# Autodesk Inventor assembly: 000.002 - Крепеж мотора СБ
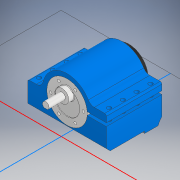
[picture p0: Inventor's stored thumbnail of the model, 180x180]
Saved by Autodesk Inventor 2022 (Build 260153000, 153)
## iProperties
Created: 2022-02-23
Part Number: 000.002 - Крепеж мотора СБ
Document SubType Name: Assembly
Designer: Petrov Ivan
Author: Petrov Ivan
## Documents named in this file (8)
- D:\IVAN\Ivan_desktop\Kvantorium\Projects\YouBotRobot\design\000.002 - Крепеж мотора СБ.iam
- D:\IVAN\Ivan_desktop\Kvantorium\Projects\YouBotRobot\design\000.002.001 - Крепеж мотора.ipt
- D:\IVAN\Ivan_desktop\Kvantorium\Projects\YouBotRobot\design\standart_components\dc_gear_motor_12V_500rpm.ipt
- D:\IVAN\Ivan_desktop\Kvantorium\Projects\YouBotRobot\design\standart_components\vex_mechanum_adapter.ipt
- D:\IVAN\Ivan_desktop\Kvantorium\Projects\YouBotRobot\design\standart_components\Rueda 1.ipt
- D:\IVAN\Ivan_desktop\Kvantorium\Projects\YouBotRobot\design\standart_components\vex_mechanum_adapter (1) зеркальный.ipt
- C:\Users\Petrov Ivan\Documents\Inventor\Content Center Files\R2022\ru-RU\CSN 02 1143  B\CSN 02 1143 - M4 x 0,7 x 40(2).ipt
- C:\Users\Petrov Ivan\Documents\Inventor\Content Center Files\R2022\ru-RU\ISO 4032(2)\ISO 4032 - M4 - ISO.ipt
## Components (19 placed, 7 different names)
1. 000.002.001 - Крепеж мотора:1 — Совмещение:1, Заподлицо:1, Угол:1
2. dc_gear_motor_12V_500rpm:1 — Совмещение:1, Заподлицо:1, Угол:1, Совмещение:2, Совмещение:3
3. vex_mechanum_adapter:1 — Совмещение:2, Совмещение:3, Совмещение:4, Совмещение:5, Совмещение:6, Совмещение:9, Совмещение:13, Совмещение:14, Совмещение:15, Заподлицо:2
4. Rueda 1:1 — Совмещение:4, Совмещение:5, Совмещение:6, Совмещение:7, Совмещение:8
5. vex_mechanum_adapter (1) зеркальный:1 — Совмещение:7, Совмещение:8, Совмещение:9, Совмещение:10, Совмещение:11, Совмещение:12
6. CSN 02 1143 B M4 x 40:1 — Совмещение:10, Совмещение:11
7. ISO 4032 M4:1 — Совмещение:12, Совмещение:13
8. CSN 02 1143 B M4 x 40:2
9. ISO 4032 M4:2
10. CSN 02 1143 B M4 x 40:3
11. ISO 4032 M4:3
12. CSN 02 1143 B M4 x 40:4
13. ISO 4032 M4:4
14. CSN 02 1143 B M4 x 40:5
15. ISO 4032 M4:5
16. CSN 02 1143 B M4 x 40:6
17. ISO 4032 M4:6
18. CSN 02 1143 B M4 x 40:7
19. ISO 4032 M4:7
## Component patterns: (7 elements, first: CSN 02 1143 B M4 x 40:1 + ISO 4032 M4:1)
## Relationships (18: Mate 15, Flush 2, Angle 1)
- Совмещение:1 [Mate]: 000.002.001 - Крепеж мотора:1 ↔ dc_gear_motor_12V_500rpm:1
- Заподлицо:1 [Flush]: 000.002.001 - Крепеж мотора:1 ↔ dc_gear_motor_12V_500rpm:1
- Угол:1 [Angle] (0 deg): 000.002.001 - Крепеж мотора:1 ↔ dc_gear_motor_12V_500rpm:1
- Совмещение:2 [Mate]: dc_gear_motor_12V_500rpm:1 ↔ vex_mechanum_adapter:1
- Совмещение:3 [Mate]: dc_gear_motor_12V_500rpm:1 ↔ vex_mechanum_adapter:1
- Совмещение:4 [Mate]: vex_mechanum_adapter:1 ↔ Rueda 1:1
- Совмещение:5 [Mate]: vex_mechanum_adapter:1 ↔ Rueda 1:1
- Совмещение:6 [Mate]: vex_mechanum_adapter:1 ↔ Rueda 1:1
- Совмещение:7 [Mate]: Rueda 1:1 ↔ vex_mechanum_adapter (1) зеркальный:1
- Совмещение:8 [Mate]: Rueda 1:1 ↔ vex_mechanum_adapter (1) зеркальный:1
- Совмещение:9 [Mate]: vex_mechanum_adapter:1 ↔ vex_mechanum_adapter (1) зеркальный:1
- Совмещение:10 [Mate]: vex_mechanum_adapter (1) зеркальный:1 ↔ CSN 02 1143 B M4 x 40:1
- Совмещение:11 [Mate]: vex_mechanum_adapter (1) зеркальный:1 ↔ CSN 02 1143 B M4 x 40:1
- Совмещение:12 [Mate]: vex_mechanum_adapter (1) зеркальный:1 ↔ ISO 4032 M4:1
- Совмещение:13 [Mate]: vex_mechanum_adapter:1 ↔ ISO 4032 M4:1
- Совмещение:14 [Mate]: vex_mechanum_adapter:1
- Совмещение:15 [Mate]: vex_mechanum_adapter:1
- Заподлицо:2 [Flush]: vex_mechanum_adapter:1
